# Autodesk Inventor assembly: Column-belt-assembly
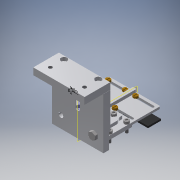
[picture p0: Inventor's stored thumbnail of the model, 180x180]
Saved by Autodesk Inventor 2016 (Build 200138000, 138)
## iProperties
Created: 2015-10-25
Part Number: Column-belt-assembly
Document SubType Name: Assembly
Designer: as
Author: as
## Documents named in this file (4)
- C:\Users\as\Documents\Inventor\mintplacer-export\export\Column-belt-assembly.iam
- C:\Users\as\Documents\Inventor\mintplacer-export\export\Portal-Column-v2.iam
- C:\Users\as\Documents\Inventor\mintplacer-export\export\belt mockup.ipt
- C:\Users\as\Documents\Inventor\mintplacer-export\export\belt-clamp-15mm-htd.ipt
## Components (3 placed, 3 different names)
1. Portal-Column-v2:1 [sub-assembly] — Mate:2, Mate:3, Mate:4
2. belt mockup:1 — Mate:2, Mate:3
3. belt-clamp-15mm-htd:1 — Mate:4
## Relationships (3: Mate 3)
- Mate:2: Portal-Column-v2:1 ↔ belt mockup:1
- Mate:3 (-25 mm): Portal-Column-v2:1 ↔ belt mockup:1
- Mate:4 (10 mm): Portal-Column-v2:1 ↔ belt-clamp-15mm-htd:1
